# Autodesk Inventor assembly: レンズ_f100
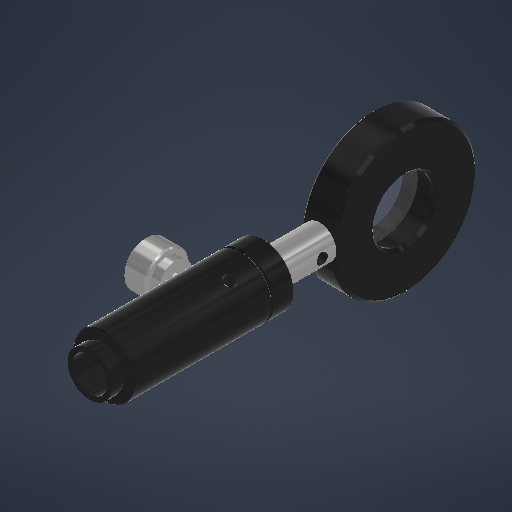
[picture p0: Inventor's stored thumbnail of the model, 512x512]
Saved by Autodesk Inventor 2026 (Build 300175050, 175E)
## iProperties
Created: 2025-07-10
Part Number: レンズ_f100
Document SubType Name: Assembly
Designer: jin20
Author: jin20
## Documents named in this file (4)
- C:\Users\jin20\Documents\装置CAD\RamanSystem\Optics\レンズ_f100.iam
- C:\Users\jin20\Documents\装置CAD\RamanSystem\Optics\レンズマウント.ipt
- C:\Users\jin20\Documents\装置CAD\RamanSystem\Optics\レンズ_f100.ipt
- C:\Users\jin20\Documents\装置CAD\RamanSystem\Optics\ロッドスタンド.ipt
## Components (3 placed, 3 different names)
1. レンズマウント:1 — 挿入:1, リジッド:1
2. レンズ_f100:1 — 挿入:1
3. ロッドスタンド:1 — リジッド:1
## Relationships (2: Insert 1, WeldJoint 1)
- 挿入:1 [Insert]: レンズマウント:1 ↔ レンズ_f100:1
- リジッド:1 [WeldJoint] (-20 mm): レンズマウント:1 ↔ ロッドスタンド:1
